# Autodesk Inventor assembly: Base
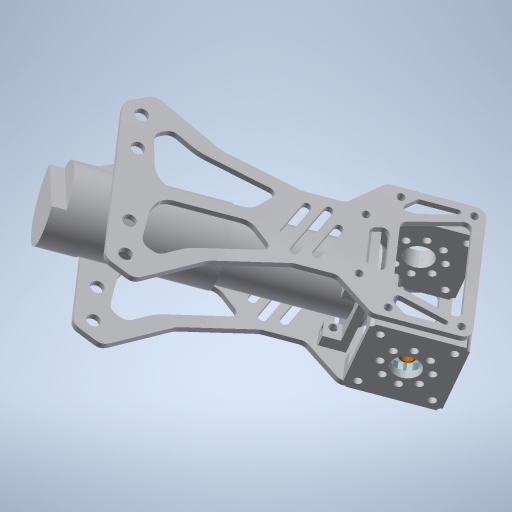
[picture p0: Inventor's stored thumbnail of the model, 512x512]
Saved by Autodesk Inventor 2023 (Build 270158000, 158)
## iProperties
Created: 2020-03-24
Part Number: Base
Document SubType Name: Assembly
Designer: valer
Mass: 715.256 g
Surface Area: 821.775 cm^2
Volume: 200.817 cm^3
Density: 3.56173 g/cm^3
Author: valer
## Documents named in this file (10)
- C:\Users\LattePanda\Desktop\str1ker\cad\ArmBase.iam
- C:\Users\LattePanda\Desktop\str1ker\cad\external\ShoulderActuator\ShoulderActuator.ipt
- C:\Users\LattePanda\Desktop\str1ker\cad\external\ShoulderMiterGear.ipt
- C:\Users\LattePanda\Desktop\str1ker\cad\external\ShoulderActuator\ShoulderActuatorShaft.ipt
- C:\Users\LattePanda\Desktop\str1ker\cad\external\ShoulderMotorMount.ipt
- C:\Users\LattePanda\Desktop\str1ker\cad\external\PatternSpacer.ipt
- C:\Users\LattePanda\Desktop\str1ker\cad\ShoulderBracket.ipt
- C:\Users\LattePanda\Desktop\str1ker\cad\external\Potentiometer\Potentiometer.iam
- C:\Users\LattePanda\Desktop\str1ker\cad\BaseBoundingBox.ipt
- C:\Users\LattePanda\Desktop\str1ker\cad\PotentiometerCover.ipt
## Components (13 placed, 9 different names)
1. ShoulderServo:1 — Mate:301, Mate:367, Mate:368
2. ShoulderMiterGear:1 — Mate:303, Mate:369
3. ShoulderServoShaft:1 — Mate:301, Mate:303, Mate:316, Mate:367
4. ShoulderMotorMount:1 — Mate:316, Mate:326, Mate:365, Mate:366, Mate:368, Mate:369
5. ShoulderMotorMount:2 — Mate:321, Mate:323, Mate:324, Mate:325, Mate:328, Mate:364, Mate:370, Mate:371
6. PatternSpacer:1 — Mate:321, Mate:363, Mate:370, Mate:371, Flush:1, Mate:375
7. ShoulderBracket:1 — Mate:323, Mate:324, Mate:325, Mate:365, Mate:366, Mate:373, Angle:3
8. ShoulderBracket:2 — Mate:326, Mate:328, Mate:359, Mate:360, Mate:361, Mate:364, Angle:4
9. ShoulderMotorMount:3 — Mate:359, Mate:360, Mate:361, Mate:372, Mate:373, Mate:374, Angle:2
10. Potentiometer:1 [sub-assembly] — Mate:372, Mate:374, Angle:2, Flush:3, Mate:376, Mate:377
11. BaseBoundingBox:1 — Flush:2, Mate:375, Angle:4
12. PotentiometerCover:1 — Flush:3
13. PotentiometerCover:2 — Mate:376, Mate:377
## Relationships (33: Mate 27, Flush 3, Angle 3)
- Mate:301: ShoulderServo:1 ↔ ShoulderServoShaft:1
- Mate:303: ShoulderMiterGear:1 ↔ ShoulderServoShaft:1
- Mate:316: ShoulderServoShaft:1 ↔ ShoulderMotorMount:1
- Mate:321: ShoulderMotorMount:2 ↔ PatternSpacer:1
- Mate:323: ShoulderMotorMount:2 ↔ ShoulderBracket:1
- Mate:324: ShoulderMotorMount:2 ↔ ShoulderBracket:1
- Mate:325: ShoulderMotorMount:2 ↔ ShoulderBracket:1
- Mate:326: ShoulderMotorMount:1 ↔ ShoulderBracket:2
- Mate:328: ShoulderMotorMount:2 ↔ ShoulderBracket:2
- Mate:359: ShoulderBracket:2 ↔ ShoulderMotorMount:3
- Mate:360: ShoulderBracket:2 ↔ ShoulderMotorMount:3
- Mate:361: ShoulderBracket:2 ↔ ShoulderMotorMount:3
- Mate:363: PatternSpacer:1
- Mate:364: ShoulderMotorMount:2 ↔ ShoulderBracket:2
- Mate:365: ShoulderMotorMount:1 ↔ ShoulderBracket:1
- Mate:366: ShoulderMotorMount:1 ↔ ShoulderBracket:1
- Mate:367 (-4 mm): ShoulderServo:1 ↔ ShoulderServoShaft:1
- Mate:368: ShoulderServo:1 ↔ ShoulderMotorMount:1
- Mate:369 (1 mm): ShoulderMiterGear:1 ↔ ShoulderMotorMount:1
- Mate:370: ShoulderMotorMount:2 ↔ PatternSpacer:1
- Mate:371: ShoulderMotorMount:2 ↔ PatternSpacer:1
- Mate:372: ShoulderMotorMount:3 ↔ Potentiometer:1
- Mate:373: ShoulderBracket:1 ↔ ShoulderMotorMount:3
- Flush:1: PatternSpacer:1
- Mate:374: ShoulderMotorMount:3 ↔ Potentiometer:1
- Angle:2 (0 deg): ShoulderMotorMount:3 ↔ Potentiometer:1
- Flush:2: BaseBoundingBox:1
- Angle:3 (0 deg): ShoulderBracket:1
- Mate:375: PatternSpacer:1 ↔ BaseBoundingBox:1
- Angle:4 (0 deg): ShoulderBracket:2 ↔ BaseBoundingBox:1
- Flush:3: Potentiometer:1 ↔ PotentiometerCover:1
- Mate:376: Potentiometer:1 ↔ PotentiometerCover:2
- Mate:377: Potentiometer:1 ↔ PotentiometerCover:2
